# Autodesk Inventor assembly: Assembly_End_Effector
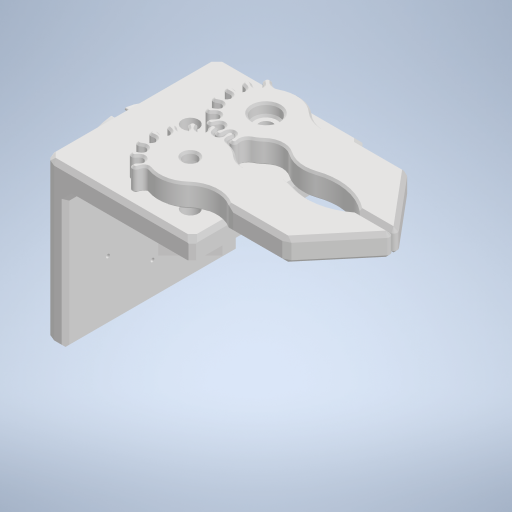
[picture p0: Inventor's stored thumbnail of the model, 512x512]
Saved by Autodesk Inventor 2023 (Build 270158000, 158)
## iProperties
Created: 2025-02-28
Part Number: Assembly_End_Effector
Document SubType Name: Assembly
Designer: Swoby
Author: Swoby
## Documents named in this file (4)
- C:\Users\Swoby\OneDrive\Plocha\Projekt\Robot_DUM-E\V0.3\Light_model\Assembly_End_Effector.iam
- C:\Users\Swoby\OneDrive\Plocha\Projekt\Robot_DUM-E\V0.3\Light_model\End_Effecto_Base.ipt
- C:\Users\Swoby\OneDrive\Plocha\Projekt\Robot_DUM-E\V0.3\Light_model\End_Effecto_Claw.ipt
- C:\Users\Swoby\OneDrive\Plocha\Projekt\Robot_DUM-E\V0.3\Light_model\End_Effecto_Claw_R.ipt
## Components (3 placed, 3 different names)
1. End_Effecto_Base:1 — Mate:1, Mate:2, Mate:3, Mate:4, Flush:1, Flush:2
2. End_Effecto_Claw:1 — Mate:1, Mate:2, Flush:1
3. End_Effecto_Claw_R:1 — Mate:3, Mate:4, Flush:2
## Relationships (6: Mate 4, Flush 2)
- Mate:1: End_Effecto_Base:1 ↔ End_Effecto_Claw:1
- Mate:2: End_Effecto_Base:1 ↔ End_Effecto_Claw:1
- Mate:3: End_Effecto_Base:1 ↔ End_Effecto_Claw_R:1
- Mate:4: End_Effecto_Base:1 ↔ End_Effecto_Claw_R:1
- Flush:1 (23 mm): End_Effecto_Base:1 ↔ End_Effecto_Claw:1
- Flush:2 (23 mm): End_Effecto_Base:1 ↔ End_Effecto_Claw_R:1
